# Autodesk Inventor assembly: handle_monitor_left
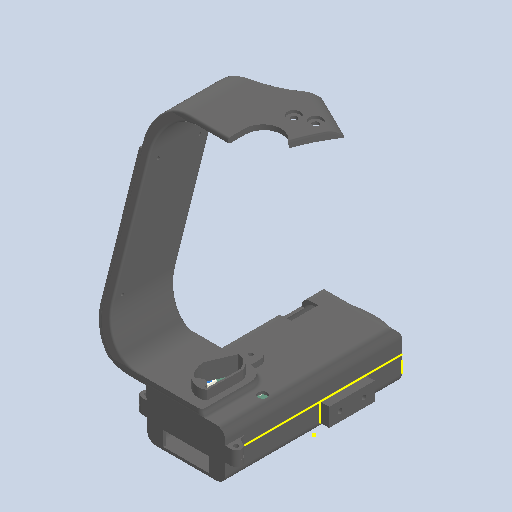
[picture p0: Inventor's stored thumbnail of the model, 512x512]
Saved by Autodesk Inventor 2026.1 (Build 301233020, 233B)
## iProperties
Created: 2026-02-03
Part Number: handle_monitor_left
Document SubType Name: Assembly
Designer: hibik
Author: hibik
## Documents named in this file (7)
- C:\Users\hibik\Documents\Robomech\HR\controller\hard\handle_left\handle_monitor_left.iam
- C:\Users\hibik\Documents\Robomech\HR\controller\hard\handle_left\handle_monitor_left.ipt
- C:\Users\hibik\Documents\Robomech\HR\controller\hard\handle_left\controller_board_left.iam
- C:\Users\hibik\Documents\Robomech\HR\controller\hard\handle_left\battery_box_left.ipt
- C:\Users\hibik\Documents\Robomech\HR\controller\hard\handle_left\handle_monitor_case_under_left.ipt
- C:\Users\hibik\Documents\Robomech\HR\controller\hard\handle_left\OLED_Display_left.iam
- C:\Users\hibik\Documents\Robomech\HR\controller\hard\handle_left\handle_monitor_case_side_left.ipt
## Components (6 placed, 6 different names)
1. handle_monitor_left:1 — 角度:1, 挿入:1, フラッシュ:3, メイト:1, フラッシュ:2, 角度:3, 挿入:3
2. controller_board_left:1 [sub-assembly] — 角度:1, 挿入:1, 角度:2, 挿入:2
3. battery_box_left:1 — 角度:2, 挿入:2
4. handle_monitor_case_under_left:1 — フラッシュ:3, メイト:1, フラッシュ:2
5. OLED_Display_left:1 [sub-assembly] — 角度:3, 挿入:3
6. handle_monitor_case_side_left:1
## Relationships (9: Angle 3, Insert 3, Flush 2, Mate 1)
- 角度:1 [Angle] (0 deg): handle_monitor_left:1 ↔ controller_board_left:1
- 挿入:1 [Insert]: handle_monitor_left:1 ↔ controller_board_left:1
- 角度:2 [Angle] (0 deg): controller_board_left:1 ↔ battery_box_left:1
- 挿入:2 [Insert]: controller_board_left:1 ↔ battery_box_left:1
- フラッシュ:3 [Flush]: handle_monitor_left:1 ↔ handle_monitor_case_under_left:1
- メイト:1 [Mate]: handle_monitor_left:1 ↔ handle_monitor_case_under_left:1
- フラッシュ:2 [Flush]: handle_monitor_left:1 ↔ handle_monitor_case_under_left:1
- 角度:3 [Angle] (0 deg): handle_monitor_left:1 ↔ OLED_Display_left:1
- 挿入:3 [Insert]: handle_monitor_left:1 ↔ OLED_Display_left:1
